# Autodesk Inventor assembly: Katze
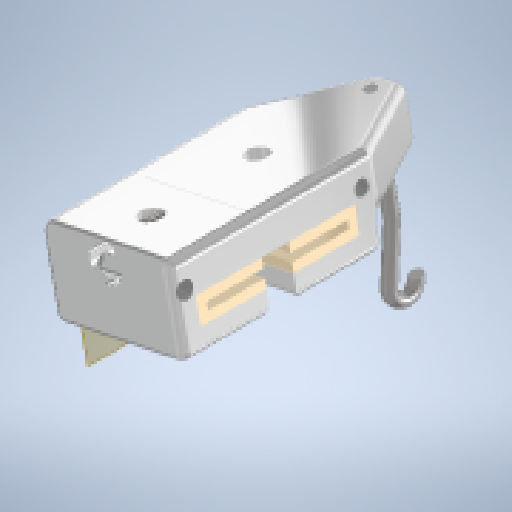
[picture p0: Inventor's stored thumbnail of the model, 512x512]
Saved by Autodesk Inventor 2025 (Build 290162010, 162A)
## iProperties
Created: 2024-11-19
Part Number: Katze
Document SubType Name: Assembly
Designer: Admin
Author: Admin
## Documents named in this file (10)
- C:\Users\Admin\GIT\HDVKBM\CAD\Krandemonstrator\Katze.iam
- C:\Users\Admin\GIT\HDVKBM\CAD\Krandemonstrator\Katze_Lagerhalter_hinten.ipt
- C:\Users\Admin\Documents\Inventor\Content Center Files\R2025\de-DE\BS 1804\BS 1804-2 - 2 x 10.ipt
- C:\Users\Admin\GIT\HDVKBM\CAD\Krandemonstrator\Katze_Lagerhalter_vorne.ipt
- C:\Users\Admin\Documents\Inventor\Content Center Files\R2025\de-DE\AS 1420\AS 1420 - 1973 - M4 x 12.ipt
- C:\Users\Admin\GIT\HDVKBM\CAD\Krandemonstrator\LagerHH.ipt
- C:\Users\Admin\Documents\Inventor\Content Center Files\R2025\de-DE\AS 1427(03)\AS 1427 - M2 x 4(1).ipt
- C:\Users\Admin\GIT\HDVKBM\CAD\Krandemonstrator\LagerHO.ipt
- C:\Users\Admin\GIT\HDVKBM\CAD\Krandemonstrator\M3 Haken 40mm.ipt
- C:\Users\Admin\Documents\Inventor\Content Center Files\R2025\de-DE\DIN 934\DIN 934 - M3 x 0,5.ipt
## Components (19 placed, 9 different names)
1. Katze_Lagerhalter_hinten:1 — Starr:7, Starr:6, Drehbar:1, Planar:1, Zylindrisch:5, Planar:2, Planar:3, Zylindrisch:6, Planar:5, Zylindrisch:7
2. BS 1804 : Teil 2 2 x 10:1 — Starr:7, Zylindrisch:4
3. BS 1804 : Teil 2 2 x 10:2 — Starr:6, Zylindrisch:3
4. Katze_Lagerhalter_vorne:1 — Zylindrisch:3, Zylindrisch:4, KatzeVH-Schraube, Planar:7, Zylindrisch:8, Planar:8, Planar:10, Zylindrisch:9, Planar:12, Zylindrisch:10, Starr:13, Einfügen:1
5. AS 1420 - Metrisch M4 x 12:1 — Drehbar:1, KatzeVH-Schraube
6. AS 1427 - Metrisch M2 x 4:1 — Starr:4, Zylindrisch:5
7. AS 1427 - Metrisch M2 x 4:2 — Starr:11, Zylindrisch:9
8. AS 1427 - Metrisch M2 x 4:3 — Starr:12, Zylindrisch:10
9. AS 1427 - Metrisch M2 x 4:4 — Starr:9, Zylindrisch:7
10. AS 1427 - Metrisch M2 x 4:5 — Starr:8, Zylindrisch:6
11. AS 1427 - Metrisch M2 x 4:6 — Starr:10, Zylindrisch:8
12. LagerHH:1 — Planar:1, Starr:4, Planar:2, Planar:4, Planar:6
13. LagerHH:2 — Planar:7, Starr:10, Planar:8, Planar:11, Planar:13
14. LagerHO:1 — Starr:11, Planar:10, Planar:11
15. LagerHO:2 — Planar:5, Starr:9, Planar:6
16. LagerHO:3 — Planar:3, Starr:8, Planar:4
17. LagerHO:4 — Starr:12, Planar:12, Planar:13
18. M3 Haken 40mm:1 — Starr:13
19. DIN 934 - ersetzt durch DIN EN 24032/28673/28674 M3:1 — Einfügen:1
## Relationships (32: PlanarJoint 12, WeldJoint 10, CylindricalJoint 8, RevoluteJoint 1, Insert 1)
- Starr:7 [WeldJoint]: Katze_Lagerhalter_hinten:1 ↔ BS 1804 : Teil 2 2 x 10:1
- Starr:6 [WeldJoint]: Katze_Lagerhalter_hinten:1 ↔ BS 1804 : Teil 2 2 x 10:2
- Zylindrisch:3 [CylindricalJoint]: BS 1804 : Teil 2 2 x 10:2 ↔ Katze_Lagerhalter_vorne:1
- Zylindrisch:4 [CylindricalJoint]: BS 1804 : Teil 2 2 x 10:1 ↔ Katze_Lagerhalter_vorne:1
- Drehbar:1 [RevoluteJoint]: Katze_Lagerhalter_hinten:1 ↔ AS 1420 - Metrisch M4 x 12:1
- KatzeVH-Schraube [WeldJoint] (0.165 mm): Katze_Lagerhalter_vorne:1 ↔ AS 1420 - Metrisch M4 x 12:1
- Planar:1: Katze_Lagerhalter_hinten:1 ↔ LagerHH:1
- Starr:4 [WeldJoint]: AS 1427 - Metrisch M2 x 4:1 ↔ LagerHH:1
- Zylindrisch:5 [CylindricalJoint]: Katze_Lagerhalter_hinten:1 ↔ AS 1427 - Metrisch M2 x 4:1
- Planar:2: Katze_Lagerhalter_hinten:1 ↔ LagerHH:1
- Planar:3: Katze_Lagerhalter_hinten:1 ↔ LagerHO:3
- Starr:8 [WeldJoint]: AS 1427 - Metrisch M2 x 4:5 ↔ LagerHO:3
- Zylindrisch:6 [CylindricalJoint]: Katze_Lagerhalter_hinten:1 ↔ AS 1427 - Metrisch M2 x 4:5
- Planar:4: LagerHH:1 ↔ LagerHO:3
- Planar:5: Katze_Lagerhalter_hinten:1 ↔ LagerHO:2
- Starr:9 [WeldJoint]: AS 1427 - Metrisch M2 x 4:4 ↔ LagerHO:2
- Zylindrisch:7 [CylindricalJoint]: Katze_Lagerhalter_hinten:1 ↔ AS 1427 - Metrisch M2 x 4:4
- Planar:6: LagerHH:1 ↔ LagerHO:2
- Planar:7: Katze_Lagerhalter_vorne:1 ↔ LagerHH:2
- Starr:10 [WeldJoint]: AS 1427 - Metrisch M2 x 4:6 ↔ LagerHH:2
- Zylindrisch:8 [CylindricalJoint]: Katze_Lagerhalter_vorne:1 ↔ AS 1427 - Metrisch M2 x 4:6
- Planar:8: Katze_Lagerhalter_vorne:1 ↔ LagerHH:2
- Starr:11 [WeldJoint]: AS 1427 - Metrisch M2 x 4:2 ↔ LagerHO:1
- Planar:10: Katze_Lagerhalter_vorne:1 ↔ LagerHO:1
- Zylindrisch:9 [CylindricalJoint]: Katze_Lagerhalter_vorne:1 ↔ AS 1427 - Metrisch M2 x 4:2
- Planar:11: LagerHH:2 ↔ LagerHO:1
- Starr:12 [WeldJoint]: AS 1427 - Metrisch M2 x 4:3 ↔ LagerHO:4
- Planar:12: Katze_Lagerhalter_vorne:1 ↔ LagerHO:4
- Zylindrisch:10 [CylindricalJoint]: Katze_Lagerhalter_vorne:1 ↔ AS 1427 - Metrisch M2 x 4:3
- Planar:13: LagerHH:2 ↔ LagerHO:4
- Starr:13 [WeldJoint]: Katze_Lagerhalter_vorne:1 ↔ M3 Haken 40mm:1
- Einfügen:1 [Insert]: Katze_Lagerhalter_vorne:1 ↔ DIN 934 - ersetzt durch DIN EN 24032/28673/28674 M3:1
